# Autodesk Inventor assembly: Assembly - Whole
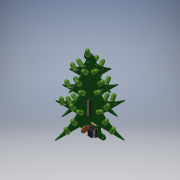
[picture p0: Inventor's stored thumbnail of the model, 180x180]
Saved by Autodesk Inventor 2018.3 (Build 223284000, 284)
## iProperties
Created: 2019-07-25
Part Number: Assembly - Whole
Document SubType Name: Assembly
Designer: Electro707
Author: Electro707
## Documents named in this file (6)
- F:\Projects\UNH MakerSpace Kits\2019 - Winter Holiday\Dual Tree Construction\GitHub Folder\CAD - Inventor\Assembly - Whole.iam
- F:\Projects\UNH MakerSpace Kits\2019 - Winter Holiday\Dual Tree Construction\GitHub Folder\CAD - Inventor\Base.ipt
- C:\Users\Electro707\Documents\Inventor\Content Center Files\R2018\en-US\BS 4183(1)\BS 4183 - M3(1).ipt
- C:\Users\Electro707\Documents\Inventor\Content Center Files\R2018\en-US\ANSI B18.6.7M(00)\ANSI B18.6.7M - M3x0.5 x 8(4).ipt
- F:\Projects\UNH MakerSpace Kits\2019 - Winter Holiday\Dual Tree Construction\GitHub Folder\CAD - Inventor\Assembly - Main Tree.iam
- F:\Projects\UNH MakerSpace Kits\2019 - Winter Holiday\Dual Tree Construction\GitHub Folder\CAD - Inventor\Assembly - Aux Tree.iam
## Components (8 placed, 5 different names)
1. Base:1 — Mate:57, Mate:58, Mate:66, Mate:67, Planar:1
2. Cross Recessed Pan Head Machine Screw - Type I - Metric M3x0.5 x 8:1 — Mate:71
3. Cross Recessed Pan Head Machine Screw - Type I - Metric M3x0.5 x 8:2 — Mate:72
4. BS 4183 - Metric M3:3 — Mate:66, Mate:68
5. BS 4183 - Metric M3:4 — Mate:67, Mate:69
6. Assembly - Main Tree:1 [sub-assembly] — Mate:71, Mate:72, Planar:1, Mate:73, Mate:74, Cylindrical:1, Cylindrical:2, Cylindrical:3, Cylindrical:4
7. Assembly - Aux Tree:1 [sub-assembly] — Mate:73, Cylindrical:3, Cylindrical:4
8. Assembly - Aux Tree:2 [sub-assembly] — Mate:74, Cylindrical:1, Cylindrical:2
## Relationships (23: Mate 18, CylindricalJoint 4, PlanarJoint 1)
- Mate:57: Base:1
- Mate:58: Base:1
- Mate:59
- [Mate]: Base:1 ↔ Cross Recessed Pan Head Machine Screw - Type I - Metric M3x0.5 x 8:1
- [Mate]: Base:1 ↔ Cross Recessed Pan Head Machine Screw - Type I - Metric M3x0.5 x 8:1
- [Mate]: Base:1 ↔ Cross Recessed Pan Head Machine Screw - Type I - Metric M3x0.5 x 8:2
- [Mate]: Base:1 ↔ Cross Recessed Pan Head Machine Screw - Type I - Metric M3x0.5 x 8:2
- [Mate]: Cross Recessed Pan Head Machine Screw - Type I - Metric M3x0.5 x 8:2 ↔ BS 4183 - Metric M3:4
- [Mate]: Cross Recessed Pan Head Machine Screw - Type I - Metric M3x0.5 x 8:1 ↔ BS 4183 - Metric M3:3
- Mate:66: Base:1 ↔ BS 4183 - Metric M3:3
- Mate:67: Base:1 ↔ BS 4183 - Metric M3:4
- Mate:68: BS 4183 - Metric M3:3
- Mate:69: BS 4183 - Metric M3:4
- Mate:70
- Mate:71: Cross Recessed Pan Head Machine Screw - Type I - Metric M3x0.5 x 8:1 ↔ Assembly - Main Tree:1
- Mate:72: Cross Recessed Pan Head Machine Screw - Type I - Metric M3x0.5 x 8:2 ↔ Assembly - Main Tree:1
- Planar:1: Base:1 ↔ Assembly - Main Tree:1
- Mate:73: Assembly - Main Tree:1 ↔ Assembly - Aux Tree:1
- Mate:74: Assembly - Main Tree:1 ↔ Assembly - Aux Tree:2
- Cylindrical:1: Assembly - Main Tree:1 ↔ Assembly - Aux Tree:2
- Cylindrical:2: Assembly - Main Tree:1 ↔ Assembly - Aux Tree:2
- Cylindrical:3: Assembly - Main Tree:1 ↔ Assembly - Aux Tree:1
- Cylindrical:4: Assembly - Main Tree:1 ↔ Assembly - Aux Tree:1
